# Autodesk Inventor assembly: Solar Panels With Holder
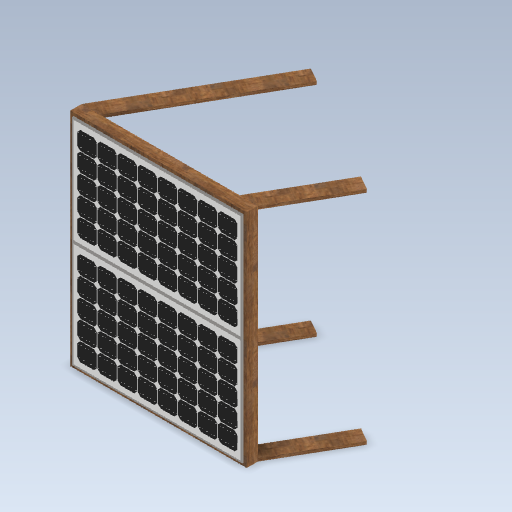
[picture p0: Inventor's stored thumbnail of the model, 512x512]
Saved by Autodesk Inventor 2020 (Build 240168000, 168)
## iProperties
Created: 2020-07-20
Part Number: Solar Panels With Holder
Document SubType Name: Assembly
Designer: Abbas
Author: Abbas
## Documents named in this file (5)
- C:\Users\LENOVO\Desktop\Graduation Project\Fish Farming Unit\Solar Panels With Holder\Solar Panels With Holder.iam
- C:\Users\LENOVO\Desktop\Graduation Project\Fish Farming Unit\solar panels holder\solar panels holder.ipt
- C:\Users\LENOVO\Desktop\Graduation Project\Fish Farming Unit\solar panel\Assembly1.iam
- C:\Users\LENOVO\Desktop\Graduation Project\Fish Farming Unit\solar panels holder\Part2.ipt
- C:\Users\LENOVO\Desktop\Graduation Project\Fish Farming Unit\solar panels holder\Part1.ipt
## Components (7 placed, 4 different names)
1. solar panels holder:2 — Mate:1, Mate:2, Mate:3, Mate:4, Mate:5, Mate:6, Mate:7, Mate:8, Mate:9, Mate:10, Mate:11, Mate:12
2. Assembly1:1 [sub-assembly] — Mate:1, Mate:2
3. Assembly1:2 [sub-assembly] — Mate:3, Mate:4
4. Part2:1 — Mate:5, Mate:6
5. Part1:1 — Mate:7, Mate:8
6. Part1:2 — Mate:9, Mate:10
7. Part2:2 — Mate:11, Mate:12
## Relationships (12: Mate 12)
- Mate:1: solar panels holder:2 ↔ Assembly1:1
- Mate:2: solar panels holder:2 ↔ Assembly1:1
- Mate:3: solar panels holder:2 ↔ Assembly1:2
- Mate:4: solar panels holder:2 ↔ Assembly1:2
- Mate:5: solar panels holder:2 ↔ Part2:1
- Mate:6: solar panels holder:2 ↔ Part2:1
- Mate:7: solar panels holder:2 ↔ Part1:1
- Mate:8: solar panels holder:2 ↔ Part1:1
- Mate:9: solar panels holder:2 ↔ Part1:2
- Mate:10: solar panels holder:2 ↔ Part1:2
- Mate:11: solar panels holder:2 ↔ Part2:2
- Mate:12: solar panels holder:2 ↔ Part2:2
